# Autodesk Inventor assembly: kill switch
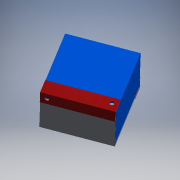
[picture p0: Inventor's stored thumbnail of the model, 180x180]
Saved by Autodesk Inventor 2019 (Build 230136000, 136)
## iProperties
Created: 2020-05-29
Part Number: kill switch
Document SubType Name: Assembly
Designer: luiza
Author: luiza
## Documents named in this file (4)
- G:\Meu Drive\Projetos\Projeto 2020 2021\Eletrônica 2020-2021\Projeção mecânica\KS\kill switch.iam
- G:\Meu Drive\Projetos\Projeto 2020 2021\Eletrônica 2020-2021\Projeção mecânica\KS\fixaçãoChaveGeral1.ipt
- G:\Meu Drive\Projetos\Projeto 2020 2021\Eletrônica 2020-2021\Projeção mecânica\KS\junção do KS .ipt
- G:\Meu Drive\Projetos\Projeto 2020 2021\Eletrônica 2020-2021\Projeção mecânica\KS\fixação chave geral.ipt
## Components (4 placed, 3 different names)
1. fixaçãoChaveGeral1:1 — Flush:1, Flush:2, Mate:2, Mate:3, Mate:5, Mate:6
2. junção do KS :1 — Mate:1, Mate:2, Mate:3
3. fixação chave geral:1 — Flush:1, Flush:2, Mate:1, Mate:4
4. junção do KS :2 — Mate:4, Mate:5, Mate:6
## Relationships (8: Mate 6, Flush 2)
- Flush:1: fixaçãoChaveGeral1:1 ↔ fixação chave geral:1
- Flush:2: fixaçãoChaveGeral1:1 ↔ fixação chave geral:1
- Mate:1: junção do KS :1 ↔ fixação chave geral:1
- Mate:2: fixaçãoChaveGeral1:1 ↔ junção do KS :1
- Mate:3: fixaçãoChaveGeral1:1 ↔ junção do KS :1
- Mate:4: fixação chave geral:1 ↔ junção do KS :2
- Mate:5: fixaçãoChaveGeral1:1 ↔ junção do KS :2
- Mate:6: fixaçãoChaveGeral1:1 ↔ junção do KS :2
